# Autodesk Inventor assembly: BasePulleyAssembly
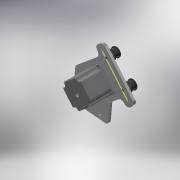
[picture p0: Inventor's stored thumbnail of the model, 180x180]
Saved by Autodesk Inventor 2020.3 (Build 243373000, 373)
## iProperties
Created: 2021-09-27
Part Number: BasePulleyAssembly
Document SubType Name: Assembly
Designer: justi
Author: justi
## Documents named in this file (5)
- F:\UQ Engineering\2021 ~ 5th Year\Semester 2\METR4911-THESIS\FarmBot CAD\FarmBotV1\BasePulleyAssembly.iam
- F:\UQ Engineering\2021 ~ 5th Year\Semester 2\METR4911-THESIS\FarmBot CAD\FarmBotV1\NEMA 23 - 56mm.iam
- F:\UQ Engineering\2021 ~ 5th Year\Semester 2\METR4911-THESIS\FarmBot CAD\FarmBotV1\GT2 Timing Pulley, Configurable, 20T W6 B5.iam
- F:\UQ Engineering\2021 ~ 5th Year\Semester 2\METR4911-THESIS\FarmBot CAD\FarmBotV1\VSlotHardware\Idler pulley kit.iam
- F:\UQ Engineering\2021 ~ 5th Year\Semester 2\METR4911-THESIS\FarmBot CAD\FarmBotV1\NEMA23MountPlatev5.ipt
## Components (5 placed, 4 different names)
1. NEMA 23 - 56mm:1 [sub-assembly] — Mate:5, Mate:6, Mate:7, Mate:8
2. GT2 Timing Pulley, Configurable, 20T W6 B5:1 [sub-assembly] — Mate:5, Flush:2
3. Idler pulley kit:2 [sub-assembly] — Flush:2, Flush:3, Mate:9
4. Idler pulley kit:3 [sub-assembly] — Flush:3, Mate:10, Flush:4
5. NEMA23MountPlatev5:1 — Mate:6, Mate:7, Mate:8, Mate:9, Mate:10, Flush:4
## Relationships (9: Mate 6, Flush 3)
- Mate:5: NEMA 23 - 56mm:1 ↔ GT2 Timing Pulley, Configurable, 20T W6 B5:1
- Flush:2: GT2 Timing Pulley, Configurable, 20T W6 B5:1 ↔ Idler pulley kit:2
- Flush:3: Idler pulley kit:2 ↔ Idler pulley kit:3
- Mate:6: NEMA 23 - 56mm:1 ↔ NEMA23MountPlatev5:1
- Mate:7: NEMA 23 - 56mm:1 ↔ NEMA23MountPlatev5:1
- Mate:8: NEMA 23 - 56mm:1 ↔ NEMA23MountPlatev5:1
- Mate:9: Idler pulley kit:2 ↔ NEMA23MountPlatev5:1
- Mate:10: Idler pulley kit:3 ↔ NEMA23MountPlatev5:1
- Flush:4: Idler pulley kit:3 ↔ NEMA23MountPlatev5:1
